# Autodesk Inventor assembly: 千斤顶
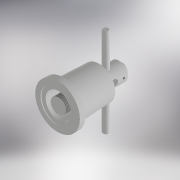
[picture p0: Inventor's stored thumbnail of the model, 180x180]
Saved by Autodesk Inventor 2020 (Build 240168000, 168)
## iProperties
Created: 2021-05-02
Part Number: 千斤顶
Document SubType Name: Assembly
Designer: Luorily
Author: Luorily
## Documents named in this file (8)
- E:\University\学习\工程图学\inventor上机-王静\千斤顶\千斤顶.iam
- E:\University\学习\工程图学\inventor上机-王静\千斤顶\底座.ipt
- E:\University\学习\工程图学\inventor上机-王静\千斤顶\螺杆.ipt
- E:\University\学习\工程图学\inventor上机-王静\千斤顶\螺套.ipt
- E:\University\学习\工程图学\inventor上机-王静\千斤顶\顶垫.ipt
- E:\University\学习\工程图学\inventor上机-王静\千斤顶\绞杆.ipt
- C:\Users\Luorily\Documents\Inventor\Content Center Files\R2020\zh-CN\GB 75-85\螺钉 GB 75-85 - M8 x 12.ipt
- C:\Users\Luorily\Documents\Inventor\Content Center Files\R2020\zh-CN\GB 73-85\螺钉 GB 73-85 - M10 x 12.ipt
## Components (7 placed, 7 different names)
1. 底座:1 — 插入:2, 插入:5, 角度:1
2. 螺杆:1 — 插入:3, 插入:4, 配合:1, 角度:1, 角度:2
3. 螺套:1 — 插入:2, 插入:3, 配合:4
4. 顶垫:1 — 插入:4, 配合:2, 配合:3, 角度:2
5. 绞杆:1 — 配合:1
6. 螺钉 GB/T 75-1985 M8 x 12:1 — 配合:2, 配合:3
7. 螺钉 GB/T 73-1985 M10 x 12:1 — 插入:5, 配合:4
## Relationships (10: Insert 4, Mate 4, Angle 2)
- 插入:2 [Insert]: 底座:1 ↔ 螺套:1
- 插入:3 [Insert]: 螺杆:1 ↔ 螺套:1
- 插入:4 [Insert]: 螺杆:1 ↔ 顶垫:1
- 配合:1 [Mate]: 螺杆:1 ↔ 绞杆:1
- 配合:2 [Mate]: 顶垫:1 ↔ 螺钉 GB/T 75-1985 M8 x 12:1
- 配合:3 [Mate]: 顶垫:1 ↔ 螺钉 GB/T 75-1985 M8 x 12:1
- 插入:5 [Insert]: 底座:1 ↔ 螺钉 GB/T 73-1985 M10 x 12:1
- 配合:4 [Mate]: 螺套:1 ↔ 螺钉 GB/T 73-1985 M10 x 12:1
- 角度:1 [Angle] (0 deg): 底座:1 ↔ 螺杆:1
- 角度:2 [Angle] (0 deg): 螺杆:1 ↔ 顶垫:1
